# Autodesk Inventor assembly: Robot Rough Outline
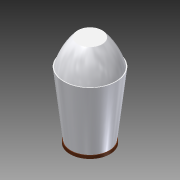
[picture p0: Inventor's stored thumbnail of the model, 180x180]
Saved by Autodesk Inventor 2014 SP2 (Build 180246200, 246)
## iProperties
Created: 2014-09-17
Part Number: Robot Rough Outline
Document SubType Name: Assembly
Designer: Sophiagirraffe
Author: Sophiagirraffe
## Documents named in this file (4)
- C:\Users\Sophiagirraffe\Dropbox\Inventor\Robot Project\Robot Rough Outline.iam
- C:\Users\Sophiagirraffe\Dropbox\Inventor\Robot Project\Trash Can Bottom.ipt
- C:\Users\Sophiagirraffe\Dropbox\Inventor\Robot Project\Head.ipt
- C:\Users\Sophiagirraffe\Dropbox\Inventor\Robot Project\Part5.ipt
## Components (3 placed, 3 different names)
1. Trash Can Bottom:1 — Rotational:1, Flush:1, Flush:2
2. Head:1 — Rotational:1
3. Part5:1 — Flush:1, Flush:2
## Relationships (3: Flush 2, RevoluteJoint 1)
- Rotational:1 [RevoluteJoint]: Trash Can Bottom:1 ↔ Head:1
- Flush:1: Trash Can Bottom:1 ↔ Part5:1
- Flush:2: Trash Can Bottom:1 ↔ Part5:1
